# Autodesk Inventor assembly: blankshortpinsPC104plus
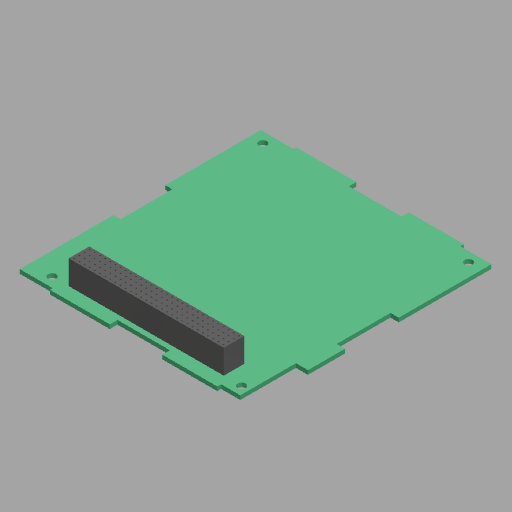
[picture p0: Inventor's stored thumbnail of the model, 512x512]
Saved by Autodesk Inventor 2022.3 (Build 263350000, 350)
## iProperties
Created: 2021-10-08
Part Number: blankshortpinsPC104plus
Document SubType Name: Assembly
Designer: Bowen O'Steen
Author: Bowen O'Steen
## Documents named in this file (3)
- C:\Users\gwhen\OneDrive\Desktop\Vault\Designs\MEMESat\MemeSat\Engineering Data\MemeSat\Subsystems\blankshortpinsPC104plus.iam
- C:\Users\gwhen\OneDrive\Desktop\Vault\Designs\MEMESat\MemeSat\Engineering Data\MemeSat\Subsystems\PC104plus.ipt
- C:\Users\gwhen\OneDrive\Desktop\Vault\Designs\MEMESat\MemeSat\Engineering Data\MemeSat\Subsystems\fullPCIshortconnector.iam
## Components (2 placed, 2 different names)
1. PC104plus:1 — Mate:1, Mate:2, Mate:3, Flush:1, Flush:2, Flush:3
2. fullPCIshortconnector:1 [sub-assembly] — Mate:1, Flush:2, Flush:3
## Relationships (6: Mate 3, Flush 3)
- Mate:1: PC104plus:1 ↔ fullPCIshortconnector:1
- Mate:2: PC104plus:1
- Mate:3: PC104plus:1
- Flush:1: PC104plus:1
- Flush:2: PC104plus:1 ↔ fullPCIshortconnector:1
- Flush:3: PC104plus:1 ↔ fullPCIshortconnector:1
